# Autodesk Inventor assembly: 20X20lift
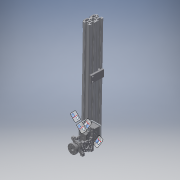
[picture p0: Inventor's stored thumbnail of the model, 180x180]
Saved by Autodesk Inventor 2017 (Build 210142000, 142)
## iProperties
Created: 2017-12-15
Part Number: 20X20lift
Document SubType Name: Assembly
Designer: User
Author: User
## Documents named in this file (11)
- C:\Robotics\CAD\2017-18_CAD\20X20lift.iam
- C:\Robotics\CAD\2017-18_CAD\Prototypes\Sliderfor2020.ipt
- C:\Robotics\CAD\COTSParts\Bosch Extrusion\Bosch 20x20 11.ipt
- C:\Robotics\CAD\2017-18_CAD\Prototypes\ServosSlideforLift.ipt
- C:\Robotics\CAD\COTSParts\Tetrix\39060_txm-standard servo bracket.ipt
- C:\Robotics\CAD\2017-18_CAD\ShoulderScrewHolderSlide.ipt
- C:\Robotics\CAD\COTSParts\Rev\REV-41-1097.ipt
- C:\Robotics\CAD\COTSParts\Actobotics\637 parts\637112\575112.ipt
- C:\Robotics\CAD\COTSParts\Actobotics\637 parts\637112\545420.ipt
- C:\Robotics\CAD\COTSParts\Actobotics\637 parts\637112\535118 assembly.ipt
- C:\Robotics\CAD\COTSParts\Actobotics\637 parts\637112\525123.ipt
## Components (14 placed, 10 different names)
1. Sliderfor2020:2 — Mate:10, Mate:11
2. Sliderfor2020:3 — Mate:5, Mate:6, Mate:8, Mate:9
3. Bosch 20x20 11:1 — Mate:5, Mate:6, Mate:11, Flush:5, Mate:25, Mate:26, Flush:8
4. Bosch 20x20 11:2 — Mate:8, Mate:9, Mate:10, Flush:5, Flush:6, Mate:21, Mate:22, Mate:23, Flush:7, Mate:24
5. ServosSlideforLift:1 — Mate:21, Mate:22, Angle:1, Insert:3
6. 39060_txm-standard servo bracket:1 — Flush:6, Insert:1, Insert:2, Angle:1, Insert:3, Mate:32, Mate:34
7. ShoulderScrewHolderSlide:1 — Mate:25, Mate:26, Flush:8
8. ShoulderScrewHolderSlide:2 — Mate:23, Flush:7, Mate:24
9. REV-41-1097:1 — Insert:1, Insert:2, Mate:31, Mate:35
10. 575112:1 — Mate:27, Flush:10, Mate:28, Flush:13, Mate:32, Mate:33, Mate:35
11. 545420:1 — Mate:27, Flush:10, Flush:12, Mate:33, Mate:34
12. 525123:1 — Mate:30, Mate:31
13. 545420:2 — Flush:12, Mate:28, Flush:13, Mate:29, Flush:15
14. 535118 assembly:1 — Mate:29, Flush:15, Mate:30
## Relationships (33: Mate 21, Flush 8, Insert 3, Angle 1)
- Mate:5: Sliderfor2020:3 ↔ Bosch 20x20 11:1
- Mate:6: Sliderfor2020:3 ↔ Bosch 20x20 11:1
- Mate:8: Sliderfor2020:3 ↔ Bosch 20x20 11:2
- Mate:9: Sliderfor2020:3 ↔ Bosch 20x20 11:2
- Mate:10: Sliderfor2020:2 ↔ Bosch 20x20 11:2
- Mate:11: Sliderfor2020:2 ↔ Bosch 20x20 11:1
- Flush:5: Bosch 20x20 11:1 ↔ Bosch 20x20 11:2
- Flush:6: Bosch 20x20 11:2 ↔ 39060_txm-standard servo bracket:1
- Mate:21: Bosch 20x20 11:2 ↔ ServosSlideforLift:1
- Mate:22: Bosch 20x20 11:2 ↔ ServosSlideforLift:1
- Insert:1: 39060_txm-standard servo bracket:1 ↔ REV-41-1097:1
- Insert:2: 39060_txm-standard servo bracket:1 ↔ REV-41-1097:1
- Angle:1 (0 deg): ServosSlideforLift:1 ↔ 39060_txm-standard servo bracket:1
- Insert:3: ServosSlideforLift:1 ↔ 39060_txm-standard servo bracket:1
- Mate:23: Bosch 20x20 11:2 ↔ ShoulderScrewHolderSlide:2
- Flush:7: Bosch 20x20 11:2 ↔ ShoulderScrewHolderSlide:2
- Mate:24 (-10 mm): Bosch 20x20 11:2 ↔ ShoulderScrewHolderSlide:2
- Mate:25: Bosch 20x20 11:1 ↔ ShoulderScrewHolderSlide:1
- Mate:26 (-10 mm): Bosch 20x20 11:1 ↔ ShoulderScrewHolderSlide:1
- Flush:8: Bosch 20x20 11:1 ↔ ShoulderScrewHolderSlide:1
- Mate:27: 575112:1 ↔ 545420:1
- Flush:10: 575112:1 ↔ 545420:1
- Flush:12: 545420:1 ↔ 545420:2
- Mate:28: 575112:1 ↔ 545420:2
- Flush:13: 575112:1 ↔ 545420:2
- Mate:29: 545420:2 ↔ 535118 assembly:1
- Flush:15: 545420:2 ↔ 535118 assembly:1
- Mate:30: 525123:1 ↔ 535118 assembly:1
- Mate:31: REV-41-1097:1 ↔ 525123:1
- Mate:32 (-7.62 mm): 39060_txm-standard servo bracket:1 ↔ 575112:1
- Mate:33: 575112:1 ↔ 545420:1
- Mate:34: 39060_txm-standard servo bracket:1 ↔ 545420:1
- Mate:35 (1.27 mm): REV-41-1097:1 ↔ 575112:1
